# Autodesk Inventor assembly: New Ripstik Assembly
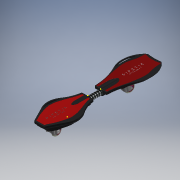
[picture p0: Inventor's stored thumbnail of the model, 180x180]
Saved by Autodesk Inventor 2018 (Build 220112000, 112)
## iProperties
Created: 2018-04-07
Part Number: New Ripstik Assembly
Document SubType Name: Assembly
Designer: Cole
Author: Cole
## Documents named in this file (7)
- P:\IED\SchoolCAD\ReverseEngineering\New Ripstik Assembly.iam
- P:\IED\SchoolCAD\ReverseEngineering\Rotation Resistor Assembly.iam
- P:\IED\SchoolCAD\ReverseEngineering\Middle Rod Assembly.iam
- P:\IED\SchoolCAD\ReverseEngineering\Wheel-Axel Assembly.iam
- P:\IED\SchoolCAD\ReverseEngineering\Double Sided Bolt Assembly.iam
- P:\IED\SchoolCAD\ReverseEngineering\New Back Board Assembly.iam
- P:\IED\SchoolCAD\ReverseEngineering\New Front Board Assembly.iam
## Components (8 placed, 6 different names)
1. Rotation Resistor Assembly:1 [sub-assembly]
2. Middle Rod Assembly:1 [sub-assembly] — Insert:10, Insert:12
3. Wheel-Axel Assembly:1 [sub-assembly] — Insert:7
4. Wheel-Axel Assembly:2 [sub-assembly] — Insert:9
5. Double Sided Bolt Assembly:1 [sub-assembly] — Insert:7, Insert:11
6. Double Sided Bolt Assembly:2 [sub-assembly] — Insert:9
7. New Back Board Assembly:1 [sub-assembly] — Insert:12
8. New Front Board Assembly:1 [sub-assembly] — Insert:10, Insert:11
## Relationships (5: Insert 5)
- Insert:7: Wheel-Axel Assembly:1 ↔ Double Sided Bolt Assembly:1
- Insert:9: Wheel-Axel Assembly:2 ↔ Double Sided Bolt Assembly:2
- Insert:10: Middle Rod Assembly:1 ↔ New Front Board Assembly:1
- Insert:11: Double Sided Bolt Assembly:1 ↔ New Front Board Assembly:1
- Insert:12: Middle Rod Assembly:1 ↔ New Back Board Assembly:1
